# Autodesk Inventor assembly: robot_rai
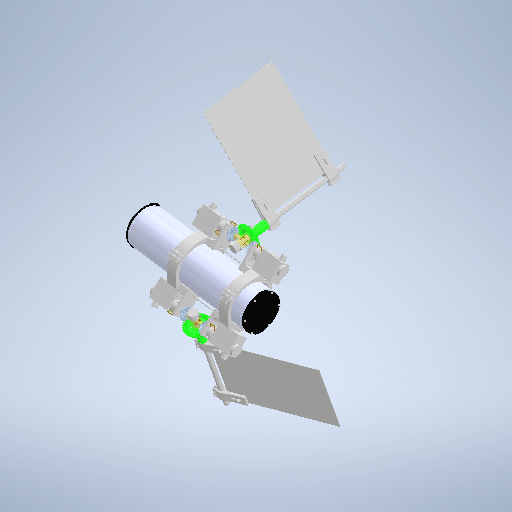
[picture p0: Inventor's stored thumbnail of the model, 512x512]
Saved by Autodesk Inventor 2025.1 (Build 291241000, 241)
## iProperties
Created: 2025-07-16
Part Number: robot_rai
Document SubType Name: Assembly
Designer: chapuzet
Author: chapuzet
## Documents named in this file (28)
- C:\Users\chapuzet\Documents\stage_ensta_rai\mecanique_robot_raie\robot_raie_voilier.iam
- C:\Users\chapuzet\Documents\stage_ensta_rai\mecanique_robot_raie\cao\pieces_finals\axe_central.ipt
- C:\Users\chapuzet\Documents\stage_ensta_rai\mecanique_robot_raie\cao\pieces_finals\attache_finaxe_central.ipt
- C:\Users\chapuzet\Documents\stage_ensta_rai\mecanique_robot_raie\cao\pieces_finals\a_usiner\bare_jonction.ipt
- C:\Users\chapuzet\Documents\stage_ensta_rai\mecanique_robot_raie\cao\pieces_finals\clamp_v2.ipt
- C:\Users\chapuzet\Documents\stage_ensta_rai\mecanique_robot_raie\cao\pieces_finals\engrenage_secondaire_v3.ipt
- C:\Users\chapuzet\Documents\stage_ensta_rai\mecanique_robot_raie\cao\pieces_finals\Cross.ipt
- C:\Users\chapuzet\Documents\stage_ensta_rai\mecanique_robot_raie\cao\pieces_finals\fixation_harbre_moteur_v2.ipt
- C:\Users\chapuzet\Documents\stage_ensta_rai\mecanique_robot_raie\cao\pieces_finals\jonction_aile_axe_centrale.ipt
- C:\Users\chapuzet\Documents\stage_ensta_rai\mecanique_robot_raie\base_meca\Servo_moteur_rovmaker_RM_SV_40.ipt
- C:\Users\chapuzet\Documents\stage_ensta_rai\mecanique_robot_raie\base_meca\pieces_bluerobotique_reference\WTE4_ACRYLIC_TUBES_BR-101052-XXX\BR-101052-300_RevB\BR-101052-300_RevB.ipt
- C:\Users\chapuzet\Documents\stage_ensta_rai\mecanique_robot_raie\cao\pieces_finals\a_usiner\aile.ipt
- C:\Users\chapuzet\Documents\stage_ensta_rai\mecanique_robot_raie\cao\pieces_finals\a_usiner\tube_carbone_mat.ipt
- C:\Users\chapuzet\Documents\stage_ensta_rai\mecanique_robot_raie\base_meca\pieces_bluerobotique_reference\WTE4_END_CAP_BLANK_BR-102993-999\WTE4-M-END-CAP-BLANK-R2\WTE4-M-END-CAP-BLANK-R2\WTE4-M-END-CAP-BLANK-R2.ipt
- C:\Users\chapuzet\Documents\stage_ensta_rai\mecanique_robot_raie\base_meca\pieces_bluerobotique_reference\WTE4_FLANGE_RAILS_BR-100665\BR-101040_RevC\BR-101040_RevC\BR-101040_RevC.ipt
- C:\Users\chapuzet\Documents\stage_ensta_rai\mecanique_robot_raie\vis\screw_gb_t_2674_m3x16_conique.ipt
- C:\Users\chapuzet\Documents\stage_ensta_rai\mecanique_robot_raie\vis\screw_gb_t_70_1_m5x35.ipt
- C:\Users\chapuzet\Documents\stage_ensta_rai\mecanique_robot_raie\vis\screw_gb_t_m3x20.ipt
- C:\Users\chapuzet\Documents\stage_ensta_rai\mecanique_robot_raie\vis\screw_gb_t_70_1_m5x25.ipt
- C:\Users\chapuzet\Documents\stage_ensta_rai\mecanique_robot_raie\vis\screw_gb_t_70_1_m4x40.ipt
- C:\Users\chapuzet\Documents\stage_ensta_rai\mecanique_robot_raie\vis\screw_gb_t_70_1_m4x12.ipt
- C:\Users\chapuzet\Documents\stage_ensta_rai\mecanique_robot_raie\vis\screw_gb_t_70_1_m4x30.ipt
- C:\Users\chapuzet\Documents\stage_ensta_rai\mecanique_robot_raie\vis\screw_gb_t_m3x35.ipt
- C:\Users\chapuzet\Documents\stage_ensta_rai\mecanique_robot_raie\vis\screw_gb_t_m3x15.ipt
- C:\Users\chapuzet\Documents\stage_ensta_rai\mecanique_robot_raie\ecrou\nut_gb_t_6170_m3.ipt
- C:\Users\chapuzet\Documents\stage_ensta_rai\mecanique_robot_raie\ecrou\nut_gb_t_6170_m5.ipt
- C:\Users\chapuzet\Documents\stage_ensta_rai\mecanique_robot_raie\ecrou\nut_gb_t_6170_m4.ipt
- C:\Users\chapuzet\Documents\stage_ensta_rai\mecanique_robot_raie\vis\tige_filte_m3x25.ipt
## Components (145 placed, 27 different names)
1. axe_central:1 — Cylindrique:7, Placage:51, Placage:67, Placage:112, Placage:113, Placage:251
2. attache_finaxe_central:1 — Placage:45, Placage:46, Placage:50, Placage:198, Placage:199, Placage:257
3. bare_jonction:1 — Placage:35, Placage:36, Cylindrique:1, Placage:41
4. bare_jonction:2 — Placage:33, Placage:34, Cylindrique:2, Placage:42
5. clamp_v2:1 — Placage:9, Placage:10, Placage:11, Placage:54, Placage:57, Placage:96, Placage:97, Placage:98, Placage:99, Placage:100, Placage:101, Placage:102, Placage:103, Placage:184, Placage:185, Placage:186, Placage:187, Placage:278, Placage:279, Placage:290, Placage:291, Placage:295
6. clamp_v2:2 — Placage:16, Placage:17, Placage:18, Placage:54, Placage:56, Placage:58, Placage:104, Placage:105, Placage:106, Placage:107, Placage:108, Placage:109, Placage:110, Placage:111, Placage:192, Placage:193, Placage:194, Placage:195, Placage:274, Placage:275, Placage:297
7. engrenage_secondaire_v3:1 — Placage:25, Placage:26, Placage:33, Placage:34
8. engrenage_secondaire_v3:2 — Placage:27, Placage:28, Placage:37, Placage:38
9. Cross:1 — Cylindrique:1, Placage:41, Cylindrique:2, Placage:42, Cylindrique:5, Placage:49, Placage:52
10. fixation_harbre_moteur_v2:1 — Placage:5, Placage:6, Placage:13, Placage:31, Placage:32, Placage:144, Placage:145, Placage:164, Placage:165, Placage:166, Placage:167, Placage:168, Placage:169, Placage:170, Placage:171, Placage:262
11. jonction_aile_axe_centrale:1 — Placage:59, Placage:67, Placage:68, Affleurement:5, Placage:79, Placage:124, Placage:125, Placage:126, Placage:127, Placage:132, Placage:135, Placage:242, Placage:243, Placage:254
12. fixation_harbre_moteur_v2:2 — Placage:3, Placage:4, Placage:14, Placage:25, Placage:26, Placage:146, Placage:147, Placage:172, Placage:173, Placage:174, Placage:175, Placage:176, Placage:177, Placage:178, Placage:179, Placage:267
13. jonction_aile_axe_centrale:2 — Placage:62, Placage:64, Affleurement:2, Placage:116, Placage:117, Placage:118, Placage:119, Placage:138, Placage:139, Placage:232, Placage:233, Placage:247
14. Servo_moteur_rovmaker_RM_SV_40:1 — Placage:7, Placage:8, Placage:15, Placage:16, Placage:17, Placage:18
15. BR-101052-300_RevB:1 — Placage:55, Placage:56, Affleurement:4, Placage:71, Placage:72, Placage:73, Placage:74
16. Servo_moteur_rovmaker_RM_SV_40:2 — Placage:1, Placage:2, Placage:9, Placage:10, Placage:11, Placage:12
17. Servo_moteur_rovmaker_RM_SV_40:4 — Placage:5, Placage:6, Placage:13, Placage:19, Placage:20, Placage:21
18. Servo_moteur_rovmaker_RM_SV_40:5 — Placage:3, Placage:4, Placage:14, Placage:22, Placage:23, Placage:24
19. clamp_v2:3 — Placage:22, Placage:23, Placage:24, Placage:53, Placage:58, Affleurement:4, Placage:88, Placage:89, Placage:90, Placage:91, Placage:92, Placage:93, Placage:94, Placage:95, Placage:188, Placage:189, Placage:190, Placage:191, Placage:282, Placage:283, Placage:299
20. clamp_v2:5 — Placage:19, Placage:20, Placage:21, Placage:53, Placage:55, Placage:57, Placage:80, Placage:81, Placage:82, Placage:83, Placage:84, Placage:85, Placage:86, Placage:87, Placage:180, Placage:181, Placage:182, Placage:183, Placage:270, Placage:271, Placage:292, Placage:293, Placage:301
21. fixation_harbre_moteur_v2:3 — Placage:7, Placage:8, Placage:15, Placage:27, Placage:28, Placage:142, Placage:143, Placage:156, Placage:157, Placage:158, Placage:159, Placage:160, Placage:161, Placage:162, Placage:163, Placage:265
22. fixation_harbre_moteur_v2:5 — Placage:1, Placage:2, Placage:12, Placage:29, Placage:30, Placage:140, Placage:141, Placage:148, Placage:149, Placage:150, Placage:151, Placage:152, Placage:153, Placage:154, Placage:155, Placage:263
23. engrenage_secondaire_v3:3 — Placage:29, Placage:30, Placage:39, Placage:40
24. engrenage_secondaire_v3:4 — Placage:31, Placage:32, Placage:35, Placage:36
25. jonction_aile_axe_centrale:3 — Placage:61, Placage:63, Placage:65, Affleurement:1, Placage:66, Placage:120, Placage:121, Placage:122, Placage:123, Placage:136, Placage:137, Placage:234, Placage:235, Placage:248
26. jonction_aile_axe_centrale:4 — Placage:60, Placage:69, Affleurement:6, Placage:128, Placage:129, Placage:130, Placage:131, Placage:133, Placage:134, Placage:240, Placage:241, Placage:255
27. bare_jonction:3 — Placage:39, Placage:40, Cylindrique:4, Placage:44
28. bare_jonction:4 — Placage:37, Placage:38, Cylindrique:3, Placage:43
29. Cross:2 — Cylindrique:3, Placage:43, Cylindrique:4, Placage:44, Cylindrique:6, Placage:50, Placage:51
30. axe_central:2 — Cylindrique:8, Placage:52, Placage:65, Placage:114, Placage:115, Placage:249
31. aile:1 — Placage:68, Placage:69, Affleurement:5, Placage:79, Affleurement:6
32. tube_carbone_mat:1 — Placage:45, Placage:46, Cylindrique:6, Cylindrique:7, Placage:59, Placage:60, Placage:285
33. aile:2 — Placage:63, Placage:64, Affleurement:1, Placage:66, Affleurement:2
34. attache_finaxe_central:2 — Placage:49, Placage:196, Placage:197, Placage:259
35. tube_carbone_mat:2 — Cylindrique:5, Cylindrique:8, Placage:61, Placage:62, Placage:289
36. WTE4-M-END-CAP-BLANK-R2:1 — Placage:76, Placage:200, Placage:201, Placage:202, Placage:203, Placage:204, Placage:205, Placage:206, Placage:207, Placage:208, Placage:209, Placage:210, Placage:211, Placage:213
37. WTE4-M-END-CAP-BLANK-R2:2 — Placage:78, Placage:214, Placage:215, Placage:216, Placage:217, Placage:218, Placage:219, Placage:221, Placage:222, Placage:223, Placage:224, Placage:225, Placage:226, Placage:227
38. BR-101040_RevC:1 — Placage:71, Placage:72, Placage:78, Placage:220, Placage:227
39. BR-101040_RevC:2 — Placage:73, Placage:74, Placage:76, Placage:212, Placage:213
40. screw_gb_t_2674_m3x16_conique:1 — Placage:83, Placage:86
41. screw_gb_t_2674_m3x16_conique:2 — Placage:81, Placage:87
42. screw_gb_t_2674_m3x16_conique:3 — Placage:82, Placage:85
43. screw_gb_t_2674_m3x16_conique:4 — Placage:80, Placage:84
44. screw_gb_t_2674_m3x16_conique:5 — Placage:90, Placage:93
45. screw_gb_t_2674_m3x16_conique:6 — Placage:88, Placage:95
46. screw_gb_t_2674_m3x16_conique:7 — Placage:91, Placage:92
47. screw_gb_t_2674_m3x16_conique:8 — Placage:89, Placage:94
48. screw_gb_t_2674_m3x16_conique:9 — Placage:99, Placage:101
49. screw_gb_t_2674_m3x16_conique:10 — Placage:97, Placage:100
50. screw_gb_t_2674_m3x16_conique:11 — Placage:98, Placage:102
51. screw_gb_t_2674_m3x16_conique:12 — Placage:96, Placage:103
52. screw_gb_t_2674_m3x16_conique:13 — Placage:107, Placage:110
53. screw_gb_t_2674_m3x16_conique:14 — Placage:105, Placage:108
54. screw_gb_t_2674_m3x16_conique:15 — Placage:106, Placage:111
55. screw_gb_t_2674_m3x16_conique:16 — Placage:104, Placage:109
56. screw_gb_t_70_1_m5x35:1 — Placage:112, Placage:113, Placage:250, Placage:284
57. screw_gb_t_70_1_m5x35:3 — Placage:114, Placage:115, Placage:246, Placage:288
58. screw_gb_t_m3x20:1 — Placage:116, Placage:118, Placage:228
59. screw_gb_t_m3x20:2 — Placage:117, Placage:119, Placage:229
60. screw_gb_t_m3x20:3 — Placage:121, Placage:122, Placage:230
61. screw_gb_t_m3x20:4 — Placage:120, Placage:123, Placage:231
62. screw_gb_t_m3x20:5 — Placage:125, Placage:127, Placage:236
63. screw_gb_t_m3x20:6 — Placage:124, Placage:126, Placage:237
64. screw_gb_t_m3x20:7 — Placage:129, Placage:130, Placage:238
65. screw_gb_t_m3x20:8 — Placage:128, Placage:131, Placage:239
66. screw_gb_t_70_1_m5x25:1 — Placage:132, Placage:135, Placage:253, Placage:286
67. screw_gb_t_70_1_m5x25:2 — Placage:133, Placage:134, Placage:252
68. screw_gb_t_70_1_m5x25:3 — Placage:136, Placage:137, Placage:244, Placage:287
69. screw_gb_t_70_1_m5x25:4 — Placage:138, Placage:139, Placage:245
70. screw_gb_t_70_1_m4x40:1 — Placage:140, Placage:141, Placage:260
71. screw_gb_t_70_1_m4x40:2 — Placage:142, Placage:143, Placage:264
72. screw_gb_t_70_1_m4x40:3 — Placage:144, Placage:145, Placage:261
73. screw_gb_t_70_1_m4x40:4 — Placage:146, Placage:147, Placage:266
74. screw_gb_t_70_1_m4x12:1 — Placage:148, Placage:155
75. screw_gb_t_70_1_m4x12:2 — Placage:149, Placage:154
76. screw_gb_t_70_1_m4x12:3 — Placage:151, Placage:153
77. screw_gb_t_70_1_m4x12:4 — Placage:150, Placage:152
78. screw_gb_t_70_1_m4x12:5 — Placage:156, Placage:160
79. screw_gb_t_70_1_m4x12:6 — Placage:159, Placage:162
80. screw_gb_t_70_1_m4x12:7 — Placage:158, Placage:163
81. screw_gb_t_70_1_m4x12:8 — Placage:157, Placage:161
82. screw_gb_t_70_1_m4x12:9 — Placage:164, Placage:166
83. screw_gb_t_70_1_m4x12:10 — Placage:165, Placage:167
84. screw_gb_t_70_1_m4x12:11 — Placage:168, Placage:170
85. screw_gb_t_70_1_m4x12:12 — Placage:169, Placage:171
86. screw_gb_t_70_1_m4x12:13 — Placage:172, Placage:173
87. screw_gb_t_70_1_m4x12:14 — Placage:174, Placage:175
88. screw_gb_t_70_1_m4x12:15 — Placage:177, Placage:179
89. screw_gb_t_70_1_m4x12:16 — Placage:176, Placage:178
90. screw_gb_t_70_1_m4x30:1 — Placage:180, Placage:183, Placage:277
91. screw_gb_t_70_1_m4x30:2 — Placage:181, Placage:182, Placage:276
92. screw_gb_t_70_1_m4x30:3 — Placage:185, Placage:187, Placage:269
93. screw_gb_t_70_1_m4x30:4 — Placage:184, Placage:186, Placage:268
94. screw_gb_t_70_1_m4x30:5 — Placage:188, Placage:190, Placage:273
95. screw_gb_t_70_1_m4x30:6 — Placage:189, Placage:191, Placage:272
96. screw_gb_t_70_1_m4x30:7 — Placage:192, Placage:194, Placage:280
97. screw_gb_t_70_1_m4x30:8 — Placage:193, Placage:195, Placage:281
98. screw_gb_t_m3x35:1 — Placage:196, Placage:197, Placage:258
99. screw_gb_t_m3x35:2 — Placage:198, Placage:199, Placage:256
100. screw_gb_t_m3x15:1 — Placage:202, Placage:211
101. screw_gb_t_m3x15:2 — Placage:200, Placage:209
102. screw_gb_t_m3x15:3 — Placage:201, Placage:210
103. screw_gb_t_m3x15:4 — Placage:203, Placage:206, Placage:212
104. screw_gb_t_m3x15:5 — Placage:204, Placage:207
105. screw_gb_t_m3x15:6 — Placage:205, Placage:208
106. screw_gb_t_m3x15:7 — Placage:214, Placage:225
107. screw_gb_t_m3x15:8 — Placage:215, Placage:224
108. screw_gb_t_m3x15:9 — Placage:216, Placage:223
109. screw_gb_t_m3x15:10 — Placage:217, Placage:226
110. screw_gb_t_m3x15:11 — Placage:218, Placage:220, Placage:221
111. screw_gb_t_m3x15:12 — Placage:219, Placage:222
112. nut_gb_t_6170_m3:1 — Placage:230, Placage:234
113. nut_gb_t_6170_m3:2 — Placage:231, Placage:235
114. nut_gb_t_6170_m3:3 — Placage:229, Placage:232
115. nut_gb_t_6170_m3:4 — Placage:228, Placage:233
116. nut_gb_t_6170_m3:5 — Placage:236, Placage:242
117. nut_gb_t_6170_m3:6 — Placage:237, Placage:243
118. nut_gb_t_6170_m3:7 — Placage:238, Placage:241
119. nut_gb_t_6170_m3:8 — Placage:239, Placage:240
120. nut_gb_t_6170_m5:1 — Placage:244, Placage:248
121. nut_gb_t_6170_m5:2 — Placage:245, Placage:247
122. nut_gb_t_6170_m5:3 — Placage:246, Placage:249
123. nut_gb_t_6170_m5:4 — Placage:250, Placage:251
124. nut_gb_t_6170_m5:5 — Placage:252, Placage:255
125. nut_gb_t_6170_m5:6 — Placage:253, Placage:254
126. nut_gb_t_6170_m3:9 — Placage:256, Placage:257
127. nut_gb_t_6170_m3:10 — Placage:258, Placage:259
128. nut_gb_t_6170_m4:1 — Placage:260, Placage:263
129. nut_gb_t_6170_m4:2 — Placage:261, Placage:262
130. nut_gb_t_6170_m4:3 — Placage:264, Placage:265
131. nut_gb_t_6170_m4:4 — Placage:266, Placage:267
132. nut_gb_t_6170_m4:5 — Placage:268, Placage:271
133. nut_gb_t_6170_m4:6 — Placage:269, Placage:270
134. nut_gb_t_6170_m4:7 — Placage:272, Placage:274
135. nut_gb_t_6170_m4:8 — Placage:273, Placage:275
136. nut_gb_t_6170_m4:9 — Placage:276, Placage:278
137. nut_gb_t_6170_m4:10 — Placage:277, Placage:279
138. nut_gb_t_6170_m4:11 — Placage:280, Placage:282
139. nut_gb_t_6170_m4:12 — Placage:281, Placage:283
140. tige_filte_m3x25:1 — Placage:290, Placage:291, Placage:294, Placage:296
141. tige_filte_m3x25:2 — Placage:292, Placage:293, Placage:298, Placage:300
142. nut_gb_t_6170_m4:13 — Placage:294, Placage:295
143. nut_gb_t_6170_m4:14 — Placage:296, Placage:297
144. nut_gb_t_6170_m4:15 — Placage:298, Placage:299
145. nut_gb_t_6170_m4:16 — Placage:300, Placage:301
## Relationships (317: Mate 298, CylindricalJoint 8, Angle 6, Flush 5)
- Placage:1 [Mate]: Servo_moteur_rovmaker_RM_SV_40:2 ↔ fixation_harbre_moteur_v2:5
- Placage:2 [Mate]: Servo_moteur_rovmaker_RM_SV_40:2 ↔ fixation_harbre_moteur_v2:5
- Placage:3 [Mate]: fixation_harbre_moteur_v2:2 ↔ Servo_moteur_rovmaker_RM_SV_40:5
- Placage:4 [Mate]: fixation_harbre_moteur_v2:2 ↔ Servo_moteur_rovmaker_RM_SV_40:5
- Placage:5 [Mate]: fixation_harbre_moteur_v2:1 ↔ Servo_moteur_rovmaker_RM_SV_40:4
- Placage:6 [Mate]: fixation_harbre_moteur_v2:1 ↔ Servo_moteur_rovmaker_RM_SV_40:4
- Placage:7 [Mate]: Servo_moteur_rovmaker_RM_SV_40:1 ↔ fixation_harbre_moteur_v2:3
- Placage:8 [Mate]: Servo_moteur_rovmaker_RM_SV_40:1 ↔ fixation_harbre_moteur_v2:3
- Placage:9 [Mate]: clamp_v2:1 ↔ Servo_moteur_rovmaker_RM_SV_40:2
- Placage:10 [Mate]: clamp_v2:1 ↔ Servo_moteur_rovmaker_RM_SV_40:2
- Placage:11 [Mate]: clamp_v2:1 ↔ Servo_moteur_rovmaker_RM_SV_40:2
- Placage:12 [Mate]: Servo_moteur_rovmaker_RM_SV_40:2 ↔ fixation_harbre_moteur_v2:5
- Placage:13 [Mate]: fixation_harbre_moteur_v2:1 ↔ Servo_moteur_rovmaker_RM_SV_40:4
- Placage:14 [Mate]: fixation_harbre_moteur_v2:2 ↔ Servo_moteur_rovmaker_RM_SV_40:5
- Placage:15 [Mate]: Servo_moteur_rovmaker_RM_SV_40:1 ↔ fixation_harbre_moteur_v2:3
- Placage:16 [Mate]: clamp_v2:2 ↔ Servo_moteur_rovmaker_RM_SV_40:1
- Placage:17 [Mate]: clamp_v2:2 ↔ Servo_moteur_rovmaker_RM_SV_40:1
- Placage:18 [Mate]: clamp_v2:2 ↔ Servo_moteur_rovmaker_RM_SV_40:1
- Placage:19 [Mate]: Servo_moteur_rovmaker_RM_SV_40:4 ↔ clamp_v2:5
- Placage:20 [Mate]: Servo_moteur_rovmaker_RM_SV_40:4 ↔ clamp_v2:5
- Placage:21 [Mate]: Servo_moteur_rovmaker_RM_SV_40:4 ↔ clamp_v2:5
- Placage:22 [Mate]: Servo_moteur_rovmaker_RM_SV_40:5 ↔ clamp_v2:3
- Placage:23 [Mate]: Servo_moteur_rovmaker_RM_SV_40:5 ↔ clamp_v2:3
- Placage:24 [Mate]: Servo_moteur_rovmaker_RM_SV_40:5 ↔ clamp_v2:3
- Placage:25 [Mate]: engrenage_secondaire_v3:1 ↔ fixation_harbre_moteur_v2:2
- Placage:26 [Mate]: engrenage_secondaire_v3:1 ↔ fixation_harbre_moteur_v2:2
- Placage:27 [Mate]: engrenage_secondaire_v3:2 ↔ fixation_harbre_moteur_v2:3
- Placage:28 [Mate]: engrenage_secondaire_v3:2 ↔ fixation_harbre_moteur_v2:3
- Placage:29 [Mate]: fixation_harbre_moteur_v2:5 ↔ engrenage_secondaire_v3:3
- Placage:30 [Mate]: fixation_harbre_moteur_v2:5 ↔ engrenage_secondaire_v3:3
- Placage:31 [Mate]: fixation_harbre_moteur_v2:1 ↔ engrenage_secondaire_v3:4
- Placage:32 [Mate]: fixation_harbre_moteur_v2:1 ↔ engrenage_secondaire_v3:4
- Placage:33 [Mate]: bare_jonction:2 ↔ engrenage_secondaire_v3:1
- Placage:34 [Mate]: bare_jonction:2 ↔ engrenage_secondaire_v3:1
- Placage:35 [Mate]: bare_jonction:1 ↔ engrenage_secondaire_v3:4
- Placage:36 [Mate]: bare_jonction:1 ↔ engrenage_secondaire_v3:4
- Placage:37 [Mate]: engrenage_secondaire_v3:2 ↔ bare_jonction:4
- Placage:38 [Mate]: engrenage_secondaire_v3:2 ↔ bare_jonction:4
- Placage:39 [Mate]: engrenage_secondaire_v3:3 ↔ bare_jonction:3
- Placage:40 [Mate]: engrenage_secondaire_v3:3 ↔ bare_jonction:3
- Cylindrique:1: bare_jonction:1 ↔ Cross:1
- Placage:41 [Mate]: bare_jonction:1 ↔ Cross:1
- Cylindrique:2: bare_jonction:2 ↔ Cross:1
- Placage:42 [Mate]: bare_jonction:2 ↔ Cross:1
- Cylindrique:3: bare_jonction:4 ↔ Cross:2
- Placage:43 [Mate]: bare_jonction:4 ↔ Cross:2
- Cylindrique:4: bare_jonction:3 ↔ Cross:2
- Placage:44 [Mate]: bare_jonction:3 ↔ Cross:2
- Placage:45 [Mate]: attache_finaxe_central:1 ↔ tube_carbone_mat:1
- Placage:46 [Mate]: attache_finaxe_central:1 ↔ tube_carbone_mat:1
- [Mate]: attache_finaxe_central:2 ↔ tube_carbone_mat:2
- [Mate]: attache_finaxe_central:2 ↔ tube_carbone_mat:2
- Cylindrique:5: Cross:1 ↔ tube_carbone_mat:2
- Placage:49 [Mate]: Cross:1 ↔ attache_finaxe_central:2
- Cylindrique:6: Cross:2 ↔ tube_carbone_mat:1
- Placage:50 [Mate]: attache_finaxe_central:1 ↔ Cross:2
- Cylindrique:7: axe_central:1 ↔ tube_carbone_mat:1
- Placage:51 [Mate]: axe_central:1 ↔ Cross:2
- Cylindrique:8: axe_central:2 ↔ tube_carbone_mat:2
- Placage:52 [Mate]: Cross:1 ↔ axe_central:2
- Placage:53 [Mate]: clamp_v2:3 ↔ clamp_v2:5
- Placage:54 [Mate]: clamp_v2:1 ↔ clamp_v2:2
- Placage:55 [Mate]: BR-101052-300_RevB:1 ↔ clamp_v2:5
- Placage:56 [Mate]: clamp_v2:2 ↔ BR-101052-300_RevB:1
- Placage:57 [Mate]: clamp_v2:1 ↔ clamp_v2:5
- Placage:58 [Mate]: clamp_v2:2 ↔ clamp_v2:3
- Placage:59 [Mate]: jonction_aile_axe_centrale:1 ↔ tube_carbone_mat:1
- Placage:60 [Mate]: jonction_aile_axe_centrale:4 ↔ tube_carbone_mat:1
- Placage:61 [Mate]: jonction_aile_axe_centrale:3 ↔ tube_carbone_mat:2
- Placage:62 [Mate]: jonction_aile_axe_centrale:2 ↔ tube_carbone_mat:2
- Placage:63 [Mate]: jonction_aile_axe_centrale:3 ↔ aile:2
- Placage:64 [Mate]: jonction_aile_axe_centrale:2 ↔ aile:2
- Placage:65 [Mate]: jonction_aile_axe_centrale:3 ↔ axe_central:2
- Affleurement:1 [Flush]: jonction_aile_axe_centrale:3 ↔ aile:2
- Placage:66 [Mate]: jonction_aile_axe_centrale:3 ↔ aile:2
- Affleurement:2 [Flush]: jonction_aile_axe_centrale:2 ↔ aile:2
- Placage:67 [Mate]: axe_central:1 ↔ jonction_aile_axe_centrale:1
- Placage:68 [Mate]: jonction_aile_axe_centrale:1 ↔ aile:1
- Placage:69 [Mate]: jonction_aile_axe_centrale:4 ↔ aile:1
- Affleurement:4 [Flush] (-30 mm): BR-101052-300_RevB:1 ↔ clamp_v2:3
- Placage:71 [Mate]: BR-101052-300_RevB:1 ↔ BR-101040_RevC:1
- Placage:72 [Mate]: BR-101052-300_RevB:1 ↔ BR-101040_RevC:1
- Placage:73 [Mate]: BR-101052-300_RevB:1 ↔ BR-101040_RevC:2
- Placage:74 [Mate]: BR-101052-300_RevB:1 ↔ BR-101040_RevC:2
- Placage:76 [Mate]: WTE4-M-END-CAP-BLANK-R2:1 ↔ BR-101040_RevC:2
- Placage:78 [Mate]: WTE4-M-END-CAP-BLANK-R2:2 ↔ BR-101040_RevC:1
- Affleurement:5 [Flush]: jonction_aile_axe_centrale:1 ↔ aile:1
- Placage:79 [Mate]: jonction_aile_axe_centrale:1 ↔ aile:1
- Affleurement:6 [Flush]: jonction_aile_axe_centrale:4 ↔ aile:1
- Placage:80 [Mate]: clamp_v2:5 ↔ screw_gb_t_2674_m3x16_conique:4
- Placage:81 [Mate]: clamp_v2:5 ↔ screw_gb_t_2674_m3x16_conique:2
- Placage:82 [Mate]: clamp_v2:5 ↔ screw_gb_t_2674_m3x16_conique:3
- Placage:83 [Mate]: clamp_v2:5 ↔ screw_gb_t_2674_m3x16_conique:1
- Placage:84 [Mate]: clamp_v2:5 ↔ screw_gb_t_2674_m3x16_conique:4
- Placage:85 [Mate]: clamp_v2:5 ↔ screw_gb_t_2674_m3x16_conique:3
- Placage:86 [Mate]: clamp_v2:5 ↔ screw_gb_t_2674_m3x16_conique:1
- Placage:87 [Mate]: clamp_v2:5 ↔ screw_gb_t_2674_m3x16_conique:2
- Placage:88 [Mate]: clamp_v2:3 ↔ screw_gb_t_2674_m3x16_conique:6
- Placage:89 [Mate]: clamp_v2:3 ↔ screw_gb_t_2674_m3x16_conique:8
- Placage:90 [Mate]: clamp_v2:3 ↔ screw_gb_t_2674_m3x16_conique:5
- Placage:91 [Mate]: clamp_v2:3 ↔ screw_gb_t_2674_m3x16_conique:7
- Placage:92 [Mate]: clamp_v2:3 ↔ screw_gb_t_2674_m3x16_conique:7
- Placage:93 [Mate]: clamp_v2:3 ↔ screw_gb_t_2674_m3x16_conique:5
- Placage:94 [Mate]: clamp_v2:3 ↔ screw_gb_t_2674_m3x16_conique:8
- Placage:95 [Mate]: clamp_v2:3 ↔ screw_gb_t_2674_m3x16_conique:6
- Placage:96 [Mate]: clamp_v2:1 ↔ screw_gb_t_2674_m3x16_conique:12
- Placage:97 [Mate]: clamp_v2:1 ↔ screw_gb_t_2674_m3x16_conique:10
- Placage:98 [Mate]: clamp_v2:1 ↔ screw_gb_t_2674_m3x16_conique:11
- Placage:99 [Mate]: clamp_v2:1 ↔ screw_gb_t_2674_m3x16_conique:9
- Placage:100 [Mate]: clamp_v2:1 ↔ screw_gb_t_2674_m3x16_conique:10
- Placage:101 [Mate]: clamp_v2:1 ↔ screw_gb_t_2674_m3x16_conique:9
- Placage:102 [Mate]: clamp_v2:1 ↔ screw_gb_t_2674_m3x16_conique:11
- Placage:103 [Mate]: clamp_v2:1 ↔ screw_gb_t_2674_m3x16_conique:12
- Placage:104 [Mate]: clamp_v2:2 ↔ screw_gb_t_2674_m3x16_conique:16
- Placage:105 [Mate]: clamp_v2:2 ↔ screw_gb_t_2674_m3x16_conique:14
- Placage:106 [Mate]: clamp_v2:2 ↔ screw_gb_t_2674_m3x16_conique:15
- Placage:107 [Mate]: clamp_v2:2 ↔ screw_gb_t_2674_m3x16_conique:13
- Placage:108 [Mate]: clamp_v2:2 ↔ screw_gb_t_2674_m3x16_conique:14
- Placage:109 [Mate]: clamp_v2:2 ↔ screw_gb_t_2674_m3x16_conique:16
- Placage:110 [Mate]: clamp_v2:2 ↔ screw_gb_t_2674_m3x16_conique:13
- Placage:111 [Mate]: clamp_v2:2 ↔ screw_gb_t_2674_m3x16_conique:15
- Placage:112 [Mate]: axe_central:1 ↔ screw_gb_t_70_1_m5x35:1
- Placage:113 [Mate] (13 mm): axe_central:1 ↔ screw_gb_t_70_1_m5x35:1
- Placage:114 [Mate]: axe_central:2 ↔ screw_gb_t_70_1_m5x35:3
- Placage:115 [Mate] (13 mm): axe_central:2 ↔ screw_gb_t_70_1_m5x35:3
- Placage:116 [Mate]: jonction_aile_axe_centrale:2 ↔ screw_gb_t_m3x20:1
- Placage:117 [Mate]: jonction_aile_axe_centrale:2 ↔ screw_gb_t_m3x20:2
- Placage:118 [Mate]: jonction_aile_axe_centrale:2 ↔ screw_gb_t_m3x20:1
- Placage:119 [Mate]: jonction_aile_axe_centrale:2 ↔ screw_gb_t_m3x20:2
- Placage:120 [Mate]: jonction_aile_axe_centrale:3 ↔ screw_gb_t_m3x20:4
- Placage:121 [Mate]: jonction_aile_axe_centrale:3 ↔ screw_gb_t_m3x20:3
- Placage:122 [Mate]: jonction_aile_axe_centrale:3 ↔ screw_gb_t_m3x20:3
- Placage:123 [Mate]: jonction_aile_axe_centrale:3 ↔ screw_gb_t_m3x20:4
- Placage:124 [Mate]: jonction_aile_axe_centrale:1 ↔ screw_gb_t_m3x20:6
- Placage:125 [Mate]: jonction_aile_axe_centrale:1 ↔ screw_gb_t_m3x20:5
- Placage:126 [Mate]: jonction_aile_axe_centrale:1 ↔ screw_gb_t_m3x20:6
- Placage:127 [Mate]: jonction_aile_axe_centrale:1 ↔ screw_gb_t_m3x20:5
- Placage:128 [Mate]: jonction_aile_axe_centrale:4 ↔ screw_gb_t_m3x20:8
- Placage:129 [Mate]: jonction_aile_axe_centrale:4 ↔ screw_gb_t_m3x20:7
- Placage:130 [Mate]: jonction_aile_axe_centrale:4 ↔ screw_gb_t_m3x20:7
- Placage:131 [Mate]: jonction_aile_axe_centrale:4 ↔ screw_gb_t_m3x20:8
- Placage:132 [Mate]: jonction_aile_axe_centrale:1 ↔ screw_gb_t_70_1_m5x25:1
- Placage:133 [Mate]: jonction_aile_axe_centrale:4 ↔ screw_gb_t_70_1_m5x25:2
- Placage:134 [Mate]: jonction_aile_axe_centrale:4 ↔ screw_gb_t_70_1_m5x25:2
- Placage:135 [Mate]: jonction_aile_axe_centrale:1 ↔ screw_gb_t_70_1_m5x25:1
- Placage:136 [Mate]: jonction_aile_axe_centrale:3 ↔ screw_gb_t_70_1_m5x25:3
- Placage:137 [Mate]: jonction_aile_axe_centrale:3 ↔ screw_gb_t_70_1_m5x25:3
- Placage:138 [Mate]: jonction_aile_axe_centrale:2 ↔ screw_gb_t_70_1_m5x25:4
- Placage:139 [Mate]: jonction_aile_axe_centrale:2 ↔ screw_gb_t_70_1_m5x25:4
- Placage:140 [Mate]: fixation_harbre_moteur_v2:5 ↔ screw_gb_t_70_1_m4x40:1
- Placage:141 [Mate] (18 mm): fixation_harbre_moteur_v2:5 ↔ screw_gb_t_70_1_m4x40:1
- Placage:142 [Mate]: fixation_harbre_moteur_v2:3 ↔ screw_gb_t_70_1_m4x40:2
- Placage:143 [Mate] (18 mm): fixation_harbre_moteur_v2:3 ↔ screw_gb_t_70_1_m4x40:2
- Placage:144 [Mate]: fixation_harbre_moteur_v2:1 ↔ screw_gb_t_70_1_m4x40:3
- Placage:145 [Mate] (18 mm): fixation_harbre_moteur_v2:1 ↔ screw_gb_t_70_1_m4x40:3
- Placage:146 [Mate]: fixation_harbre_moteur_v2:2 ↔ screw_gb_t_70_1_m4x40:4
- Placage:147 [Mate] (18 mm): fixation_harbre_moteur_v2:2 ↔ screw_gb_t_70_1_m4x40:4
- Placage:148 [Mate]: fixation_harbre_moteur_v2:5 ↔ screw_gb_t_70_1_m4x12:1
- Placage:149 [Mate]: fixation_harbre_moteur_v2:5 ↔ screw_gb_t_70_1_m4x12:2
- Placage:150 [Mate]: fixation_harbre_moteur_v2:5 ↔ screw_gb_t_70_1_m4x12:4
- Placage:151 [Mate]: fixation_harbre_moteur_v2:5 ↔ screw_gb_t_70_1_m4x12:3
- Placage:152 [Mate]: fixation_harbre_moteur_v2:5 ↔ screw_gb_t_70_1_m4x12:4
- Placage:153 [Mate]: fixation_harbre_moteur_v2:5 ↔ screw_gb_t_70_1_m4x12:3
- Placage:154 [Mate]: fixation_harbre_moteur_v2:5 ↔ screw_gb_t_70_1_m4x12:2
- Placage:155 [Mate]: fixation_harbre_moteur_v2:5 ↔ screw_gb_t_70_1_m4x12:1
- Placage:156 [Mate]: fixation_harbre_moteur_v2:3 ↔ screw_gb_t_70_1_m4x12:5
- Placage:157 [Mate]: fixation_harbre_moteur_v2:3 ↔ screw_gb_t_70_1_m4x12:8
- Placage:158 [Mate]: fixation_harbre_moteur_v2:3 ↔ screw_gb_t_70_1_m4x12:7
- Placage:159 [Mate]: fixation_harbre_moteur_v2:3 ↔ screw_gb_t_70_1_m4x12:6
- Placage:160 [Mate]: fixation_harbre_moteur_v2:3 ↔ screw_gb_t_70_1_m4x12:5
- Placage:161 [Mate]: fixation_harbre_moteur_v2:3 ↔ screw_gb_t_70_1_m4x12:8
- Placage:162 [Mate]: fixation_harbre_moteur_v2:3 ↔ screw_gb_t_70_1_m4x12:6
- Placage:163 [Mate]: fixation_harbre_moteur_v2:3 ↔ screw_gb_t_70_1_m4x12:7
- Placage:164 [Mate]: fixation_harbre_moteur_v2:1 ↔ screw_gb_t_70_1_m4x12:9
- Placage:165 [Mate]: fixation_harbre_moteur_v2:1 ↔ screw_gb_t_70_1_m4x12:10
- Placage:166 [Mate]: fixation_harbre_moteur_v2:1 ↔ screw_gb_t_70_1_m4x12:9
- Placage:167 [Mate]: fixation_harbre_moteur_v2:1 ↔ screw_gb_t_70_1_m4x12:10
- Placage:168 [Mate]: fixation_harbre_moteur_v2:1 ↔ screw_gb_t_70_1_m4x12:11
- Placage:169 [Mate]: fixation_harbre_moteur_v2:1 ↔ screw_gb_t_70_1_m4x12:12
- Placage:170 [Mate]: fixation_harbre_moteur_v2:1 ↔ screw_gb_t_70_1_m4x12:11
- Placage:171 [Mate]: fixation_harbre_moteur_v2:1 ↔ screw_gb_t_70_1_m4x12:12
- Placage:172 [Mate]: fixation_harbre_moteur_v2:2 ↔ screw_gb_t_70_1_m4x12:13
- Placage:173 [Mate]: fixation_harbre_moteur_v2:2 ↔ screw_gb_t_70_1_m4x12:13
- Placage:174 [Mate]: fixation_harbre_moteur_v2:2 ↔ screw_gb_t_70_1_m4x12:14
- Placage:175 [Mate]: fixation_harbre_moteur_v2:2 ↔ screw_gb_t_70_1_m4x12:14
- Placage:176 [Mate]: fixation_harbre_moteur_v2:2 ↔ screw_gb_t_70_1_m4x12:16
- Placage:177 [Mate]: fixation_harbre_moteur_v2:2 ↔ screw_gb_t_70_1_m4x12:15
- Placage:178 [Mate]: fixation_harbre_moteur_v2:2 ↔ screw_gb_t_70_1_m4x12:16
- Placage:179 [Mate]: fixation_harbre_moteur_v2:2 ↔ screw_gb_t_70_1_m4x12:15
- Placage:180 [Mate]: clamp_v2:5 ↔ screw_gb_t_70_1_m4x30:1
- Placage:181 [Mate]: clamp_v2:5 ↔ screw_gb_t_70_1_m4x30:2
- Placage:182 [Mate]: clamp_v2:5 ↔ screw_gb_t_70_1_m4x30:2
- Placage:183 [Mate]: clamp_v2:5 ↔ screw_gb_t_70_1_m4x30:1
- Placage:184 [Mate]: clamp_v2:1 ↔ screw_gb_t_70_1_m4x30:4
- Placage:185 [Mate]: clamp_v2:1 ↔ screw_gb_t_70_1_m4x30:3
- Placage:186 [Mate]: clamp_v2:1 ↔ screw_gb_t_70_1_m4x30:4
- Placage:187 [Mate]: clamp_v2:1 ↔ screw_gb_t_70_1_m4x30:3
- Placage:188 [Mate]: clamp_v2:3 ↔ screw_gb_t_70_1_m4x30:5
- Placage:189 [Mate]: clamp_v2:3 ↔ screw_gb_t_70_1_m4x30:6
- Placage:190 [Mate]: clamp_v2:3 ↔ screw_gb_t_70_1_m4x30:5
- Placage:191 [Mate]: clamp_v2:3 ↔ screw_gb_t_70_1_m4x30:6
- Placage:192 [Mate]: clamp_v2:2 ↔ screw_gb_t_70_1_m4x30:7
- Placage:193 [Mate]: clamp_v2:2 ↔ screw_gb_t_70_1_m4x30:8
- Placage:194 [Mate]: clamp_v2:2 ↔ screw_gb_t_70_1_m4x30:7
- Placage:195 [Mate]: clamp_v2:2 ↔ screw_gb_t_70_1_m4x30:8
- Placage:196 [Mate]: attache_finaxe_central:2 ↔ screw_gb_t_m3x35:1
- Placage:197 [Mate] (14 mm): attache_finaxe_central:2 ↔ screw_gb_t_m3x35:1
- Placage:198 [Mate]: attache_finaxe_central:1 ↔ screw_gb_t_m3x35:2
- Placage:199 [Mate] (14 mm): attache_finaxe_central:1 ↔ screw_gb_t_m3x35:2
- Placage:200 [Mate]: WTE4-M-END-CAP-BLANK-R2:1 ↔ screw_gb_t_m3x15:2
- Placage:201 [Mate]: WTE4-M-END-CAP-BLANK-R2:1 ↔ screw_gb_t_m3x15:3
- Placage:202 [Mate]: WTE4-M-END-CAP-BLANK-R2:1 ↔ screw_gb_t_m3x15:1
- Placage:203 [Mate]: WTE4-M-END-CAP-BLANK-R2:1 ↔ screw_gb_t_m3x15:4
- Placage:204 [Mate]: WTE4-M-END-CAP-BLANK-R2:1 ↔ screw_gb_t_m3x15:5
- Placage:205 [Mate]: WTE4-M-END-CAP-BLANK-R2:1 ↔ screw_gb_t_m3x15:6
- Placage:206 [Mate]: WTE4-M-END-CAP-BLANK-R2:1 ↔ screw_gb_t_m3x15:4
- Placage:207 [Mate]: WTE4-M-END-CAP-BLANK-R2:1 ↔ screw_gb_t_m3x15:5
- Placage:208 [Mate]: WTE4-M-END-CAP-BLANK-R2:1 ↔ screw_gb_t_m3x15:6
- Placage:209 [Mate]: WTE4-M-END-CAP-BLANK-R2:1 ↔ screw_gb_t_m3x15:2
- Placage:210 [Mate]: WTE4-M-END-CAP-BLANK-R2:1 ↔ screw_gb_t_m3x15:3
- Placage:211 [Mate]: WTE4-M-END-CAP-BLANK-R2:1 ↔ screw_gb_t_m3x15:1
- Placage:212 [Mate]: BR-101040_RevC:2 ↔ screw_gb_t_m3x15:4
- Placage:213 [Mate]: WTE4-M-END-CAP-BLANK-R2:1 ↔ BR-101040_RevC:2
- Placage:214 [Mate]: WTE4-M-END-CAP-BLANK-R2:2 ↔ screw_gb_t_m3x15:7
- Placage:215 [Mate]: WTE4-M-END-CAP-BLANK-R2:2 ↔ screw_gb_t_m3x15:8
- Placage:216 [Mate]: WTE4-M-END-CAP-BLANK-R2:2 ↔ screw_gb_t_m3x15:9
- Placage:217 [Mate]: WTE4-M-END-CAP-BLANK-R2:2 ↔ screw_gb_t_m3x15:10
- Placage:218 [Mate]: WTE4-M-END-CAP-BLANK-R2:2 ↔ screw_gb_t_m3x15:11
- Placage:219 [Mate]: WTE4-M-END-CAP-BLANK-R2:2 ↔ screw_gb_t_m3x15:12
- Placage:220 [Mate]: BR-101040_RevC:1 ↔ screw_gb_t_m3x15:11
- Placage:221 [Mate]: WTE4-M-END-CAP-BLANK-R2:2 ↔ screw_gb_t_m3x15:11
- Placage:222 [Mate]: WTE4-M-END-CAP-BLANK-R2:2 ↔ screw_gb_t_m3x15:12
- Placage:223 [Mate]: WTE4-M-END-CAP-BLANK-R2:2 ↔ screw_gb_t_m3x15:9
- Placage:224 [Mate]: WTE4-M-END-CAP-BLANK-R2:2 ↔ screw_gb_t_m3x15:8
- Placage:225 [Mate]: WTE4-M-END-CAP-BLANK-R2:2 ↔ screw_gb_t_m3x15:7
- Placage:226 [Mate]: WTE4-M-END-CAP-BLANK-R2:2 ↔ screw_gb_t_m3x15:10
- Placage:227 [Mate]: WTE4-M-END-CAP-BLANK-R2:2 ↔ BR-101040_RevC:1
- Placage:228 [Mate]: screw_gb_t_m3x20:1 ↔ nut_gb_t_6170_m3:4
- Placage:229 [Mate]: screw_gb_t_m3x20:2 ↔ nut_gb_t_6170_m3:3
- Placage:230 [Mate]: screw_gb_t_m3x20:3 ↔ nut_gb_t_6170_m3:1
- Placage:231 [Mate]: screw_gb_t_m3x20:4 ↔ nut_gb_t_6170_m3:2
- Placage:232 [Mate]: jonction_aile_axe_centrale:2 ↔ nut_gb_t_6170_m3:3
- Placage:233 [Mate]: jonction_aile_axe_centrale:2 ↔ nut_gb_t_6170_m3:4
- Placage:234 [Mate]: jonction_aile_axe_centrale:3 ↔ nut_gb_t_6170_m3:1
- Placage:235 [Mate]: jonction_aile_axe_centrale:3 ↔ nut_gb_t_6170_m3:2
- Placage:236 [Mate]: screw_gb_t_m3x20:5 ↔ nut_gb_t_6170_m3:5
- Placage:237 [Mate]: screw_gb_t_m3x20:6 ↔ nut_gb_t_6170_m3:6
- Placage:238 [Mate]: screw_gb_t_m3x20:7 ↔ nut_gb_t_6170_m3:7
- Placage:239 [Mate]: screw_gb_t_m3x20:8 ↔ nut_gb_t_6170_m3:8
- Placage:240 [Mate]: jonction_aile_axe_centrale:4 ↔ nut_gb_t_6170_m3:8
- Placage:241 [Mate]: jonction_aile_axe_centrale:4 ↔ nut_gb_t_6170_m3:7
- Placage:242 [Mate]: jonction_aile_axe_centrale:1 ↔ nut_gb_t_6170_m3:5
- Placage:243 [Mate]: jonction_aile_axe_centrale:1 ↔ nut_gb_t_6170_m3:6
- Placage:244 [Mate]: screw_gb_t_70_1_m5x25:3 ↔ nut_gb_t_6170_m5:1
- Placage:245 [Mate]: screw_gb_t_70_1_m5x25:4 ↔ nut_gb_t_6170_m5:2
- Placage:246 [Mate]: screw_gb_t_70_1_m5x35:3 ↔ nut_gb_t_6170_m5:3
- Placage:247 [Mate]: jonction_aile_axe_centrale:2 ↔ nut_gb_t_6170_m5:2
- Placage:248 [Mate]: jonction_aile_axe_centrale:3 ↔ nut_gb_t_6170_m5:1
- Placage:249 [Mate] (13 mm): axe_central:2 ↔ nut_gb_t_6170_m5:3
- Placage:250 [Mate]: screw_gb_t_70_1_m5x35:1 ↔ nut_gb_t_6170_m5:4
- Placage:251 [Mate] (13 mm): axe_central:1 ↔ nut_gb_t_6170_m5:4
- Placage:252 [Mate]: screw_gb_t_70_1_m5x25:2 ↔ nut_gb_t_6170_m5:5
- Placage:253 [Mate]: screw_gb_t_70_1_m5x25:1 ↔ nut_gb_t_6170_m5:6
- Placage:254 [Mate]: jonction_aile_axe_centrale:1 ↔ nut_gb_t_6170_m5:6
- Placage:255 [Mate]: jonction_aile_axe_centrale:4 ↔ nut_gb_t_6170_m5:5
- Placage:256 [Mate]: screw_gb_t_m3x35:2 ↔ nut_gb_t_6170_m3:9
- Placage:257 [Mate] (14 mm): attache_finaxe_central:1 ↔ nut_gb_t_6170_m3:9
- Placage:258 [Mate]: screw_gb_t_m3x35:1 ↔ nut_gb_t_6170_m3:10
- Placage:259 [Mate] (14 mm): attache_finaxe_central:2 ↔ nut_gb_t_6170_m3:10
- Placage:260 [Mate]: screw_gb_t_70_1_m4x40:1 ↔ nut_gb_t_6170_m4:1
- Placage:261 [Mate]: screw_gb_t_70_1_m4x40:3 ↔ nut_gb_t_6170_m4:2
- Placage:262 [Mate] (18 mm): fixation_harbre_moteur_v2:1 ↔ nut_gb_t_6170_m4:2
- Placage:263 [Mate] (18 mm): fixation_harbre_moteur_v2:5 ↔ nut_gb_t_6170_m4:1
- Placage:264 [Mate]: screw_gb_t_70_1_m4x40:2 ↔ nut_gb_t_6170_m4:3
- Placage:265 [Mate] (18 mm): fixation_harbre_moteur_v2:3 ↔ nut_gb_t_6170_m4:3
- Placage:266 [Mate]: screw_gb_t_70_1_m4x40:4 ↔ nut_gb_t_6170_m4:4
- Placage:267 [Mate] (18 mm): fixation_harbre_moteur_v2:2 ↔ nut_gb_t_6170_m4:4
- Placage:268 [Mate]: screw_gb_t_70_1_m4x30:4 ↔ nut_gb_t_6170_m4:5
- Placage:269 [Mate]: screw_gb_t_70_1_m4x30:3 ↔ nut_gb_t_6170_m4:6
- Placage:270 [Mate]: clamp_v2:5 ↔ nut_gb_t_6170_m4:6
- Placage:271 [Mate]: clamp_v2:5 ↔ nut_gb_t_6170_m4:5
- Placage:272 [Mate]: screw_gb_t_70_1_m4x30:6 ↔ nut_gb_t_6170_m4:7
- Placage:273 [Mate]: screw_gb_t_70_1_m4x30:5 ↔ nut_gb_t_6170_m4:8
- Placage:274 [Mate]: clamp_v2:2 ↔ nut_gb_t_6170_m4:7
- Placage:275 [Mate]: clamp_v2:2 ↔ nut_gb_t_6170_m4:8
- Placage:276 [Mate]: screw_gb_t_70_1_m4x30:2 ↔ nut_gb_t_6170_m4:9
- Placage:277 [Mate]: screw_gb_t_70_1_m4x30:1 ↔ nut_gb_t_6170_m4:10
- Placage:278 [Mate]: clamp_v2:1 ↔ nut_gb_t_6170_m4:9
- Placage:279 [Mate]: clamp_v2:1 ↔ nut_gb_t_6170_m4:10
- Placage:280 [Mate]: screw_gb_t_70_1_m4x30:7 ↔ nut_gb_t_6170_m4:11
- Placage:281 [Mate]: screw_gb_t_70_1_m4x30:8 ↔ nut_gb_t_6170_m4:12
- Placage:282 [Mate]: clamp_v2:3 ↔ nut_gb_t_6170_m4:11
- Placage:283 [Mate]: clamp_v2:3 ↔ nut_gb_t_6170_m4:12
- Placage:284 [Mate]: screw_gb_t_70_1_m5x35:1
- Placage:285 [Mate]: tube_carbone_mat:1
- Angle:1 (90 deg)
- Placage:286 [Mate]: screw_gb_t_70_1_m5x25:1
- Angle:2 (90 deg)
- Angle:3 (90 deg)
- Placage:287 [Mate]: screw_gb_t_70_1_m5x25:3
- Placage:288 [Mate]: screw_gb_t_70_1_m5x35:3
- Angle:4 (90 deg)
- Placage:289 [Mate]: tube_carbone_mat:2
- Angle:5 (90 deg)
- Angle:6 (90 deg)
- Placage:290 [Mate]: clamp_v2:1 ↔ tige_filte_m3x25:1
- Placage:291 [Mate] (13 mm): clamp_v2:1 ↔ tige_filte_m3x25:1
- Placage:292 [Mate]: clamp_v2:5 ↔ tige_filte_m3x25:2
- Placage:293 [Mate] (13 mm): clamp_v2:5 ↔ tige_filte_m3x25:2
- Placage:294 [Mate]: tige_filte_m3x25:1 ↔ nut_gb_t_6170_m4:13
- Placage:295 [Mate]: clamp_v2:1 ↔ nut_gb_t_6170_m4:13
- Placage:296 [Mate]: tige_filte_m3x25:1 ↔ nut_gb_t_6170_m4:14
- Placage:297 [Mate]: clamp_v2:2 ↔ nut_gb_t_6170_m4:14
- Placage:298 [Mate]: tige_filte_m3x25:2 ↔ nut_gb_t_6170_m4:15
- Placage:299 [Mate]: clamp_v2:3 ↔ nut_gb_t_6170_m4:15
- Placage:300 [Mate]: tige_filte_m3x25:2 ↔ nut_gb_t_6170_m4:16
- Placage:301 [Mate]: clamp_v2:5 ↔ nut_gb_t_6170_m4:16
## Named parameters: d56_d54 = 0 mm, d57_d55 = 0 mm
